# Autodesk Inventor assembly: RoArm_brazo
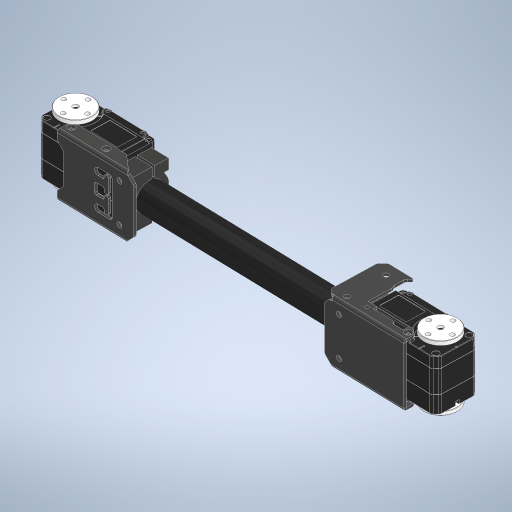
[picture p0: Inventor's stored thumbnail of the model, 512x512]
Saved by Autodesk Inventor 2024.4 (Build 284460000, 460)
## iProperties
Created: 2026-06-03
Part Number: RoArm_brazo
Document SubType Name: Assembly
Designer: epm01
Author: epm01
## Documents named in this file (6)
- D:\Archivos\2026-2\RoArm\inventor\RoArm_brazo.iam
- D:\Archivos\2026-2\RoArm\inventor\ST3215 v1\ST3215 v1\ST3215 v1.iam
- D:\Archivos\2026-2\RoArm\inventor\AL-ELBOW-B\AL-ELBOW-B\AL-ELBOW-B.ipt
- D:\Archivos\2026-2\RoArm\inventor\LEG-HOLDER v2\LEG-HOLDER v2\LEG-HOLDER v2.ipt
- D:\Archivos\2026-2\RoArm\inventor\16-140 v2\16-140 v2\16-140 v2.ipt
- D:\Archivos\2026-2\RoArm\inventor\AL-muneca\AL-muneca\AL-muneca.ipt
## Components (7 placed, 5 different names)
1. ST3215 v1:1 [sub-assembly] — Insert:1, Insert:2
2. AL-ELBOW-B:1 — Insert:1, Insert:2, Insert:3, Insert:4
3. LEG-HOLDER v2:1 — Insert:3, Insert:4, Insert:5, Flush:1
4. 16-140 v2:1 — Insert:5, Insert:6
5. LEG-HOLDER v2:2 — Insert:6, Flush:1, Insert:7, Insert:8
6. AL-muneca:1 — Insert:7, Insert:8, Insert:9, Flush:2
7. ST3215 v1:2 [sub-assembly] — Insert:9, Flush:2
## Relationships (11: Insert 9, Flush 2)
- Insert:1: ST3215 v1:1 ↔ AL-ELBOW-B:1
- Insert:2: ST3215 v1:1 ↔ AL-ELBOW-B:1
- Insert:3: AL-ELBOW-B:1 ↔ LEG-HOLDER v2:1
- Insert:4: AL-ELBOW-B:1 ↔ LEG-HOLDER v2:1
- Insert:5: LEG-HOLDER v2:1 ↔ 16-140 v2:1
- Insert:6: 16-140 v2:1 ↔ LEG-HOLDER v2:2
- Flush:1: LEG-HOLDER v2:1 ↔ LEG-HOLDER v2:2
- Insert:7: LEG-HOLDER v2:2 ↔ AL-muneca:1
- Insert:8: LEG-HOLDER v2:2 ↔ AL-muneca:1
- Insert:9: AL-muneca:1 ↔ ST3215 v1:2
- Flush:2: AL-muneca:1 ↔ ST3215 v1:2
